# Autodesk Inventor assembly: アーム先端シールド1
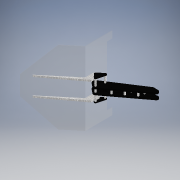
[picture p0: Inventor's stored thumbnail of the model, 180x180]
Saved by Autodesk Inventor 2020 (Build 240168000, 168)
## iProperties
Created: 2019-09-18
Part Number: アーム先端シールド1
Document SubType Name: Assembly
Designer: 雪村
Author: 雪村
## Documents named in this file (8)
- C:\Users\white\Documents\SRDC\SRDC\Inventor_2017\2018年機体\2020年4年機体\アーム先端シールド1.iam
- C:\Users\white\Documents\SRDC\SRDC\Inventor_2017\2018年機体\2020年4年機体\アーム先端第1関節2.1.ipt
- C:\Users\white\Documents\SRDC\SRDC\Inventor_2017\2018年機体\2020年4年機体\アーム先端第1関節2.1_MIR.ipt
- C:\Users\white\Documents\SRDC\SRDC\Inventor_2017\2018年機体\パーツ\スペーサーm3,16.ipt
- C:\Users\white\Documents\SRDC\SRDC\Inventor_2017\2018年機体\2020年4年機体\アームシールド根本1.ipt
- C:\Users\white\Documents\SRDC\SRDC\Inventor_2017\2018年機体\2020年4年機体\アームシールド2.ipt
- C:\Users\white\Documents\SRDC\SRDC\Inventor_2017\2018年機体\パーツ\スペーサーm3,25.ipt
- C:\Users\white\Documents\SRDC\SRDC\Inventor_2017\2018年機体\2020年4年機体\アーム抑えツイン1.ipt
## Components (22 placed, 7 different names)
1. アーム先端第1関節2.1:1 — 挿入:10, 挿入:11, 挿入:17, 挿入:18, 挿入:21
2. アーム先端第1関節2.1_MIR:1 — 挿入:1, 挿入:2, 挿入:3, 挿入:4, 挿入:5, 挿入:6, 挿入:7, 挿入:8, 挿入:9, 挿入:16, 挿入:19, 挿入:20, 挿入:22
3. スペーサーm3,16:1 — 挿入:2
4. スペーサーm3,16:2 — 挿入:1, 挿入:10
5. スペーサーm3,16:3 — 挿入:3
6. スペーサーm3,16:4 — 挿入:4
7. スペーサーm3,16:5 — 挿入:5
8. スペーサーm3,16:6 — 挿入:7
9. スペーサーm3,16:7 — 挿入:8
10. スペーサーm3,16:8 — 挿入:9
11. スペーサーm3,16:9 — 挿入:6, 挿入:11
12. アームシールド根本1:1 — 挿入:14, 挿入:15
13. アームシールド2:1 — 挿入:12, 挿入:13, 挿入:14, 挿入:15
14. アームシールド根本1:2 — 挿入:12, 挿入:13, 挿入:16
15. スペーサーm3,25:1 — 挿入:17, 挿入:25
16. スペーサーm3,25:2 — 挿入:18
17. スペーサーm3,25:3 — 挿入:19, 挿入:23
18. スペーサーm3,25:4 — 挿入:20
19. スペーサーm3,25:5 — 挿入:22, 挿入:24
20. スペーサーm3,25:6 — 挿入:21, 挿入:26
21. アーム抑えツイン1:1 — 挿入:25, 挿入:26
22. アーム抑えツイン1:2 — 挿入:23, 挿入:24
## Relationships (26: Insert 26)
- 挿入:1 [Insert]: アーム先端第1関節2.1_MIR:1 ↔ スペーサーm3,16:2
- 挿入:2 [Insert]: アーム先端第1関節2.1_MIR:1 ↔ スペーサーm3,16:1
- 挿入:3 [Insert]: アーム先端第1関節2.1_MIR:1 ↔ スペーサーm3,16:3
- 挿入:4 [Insert]: アーム先端第1関節2.1_MIR:1 ↔ スペーサーm3,16:4
- 挿入:5 [Insert]: アーム先端第1関節2.1_MIR:1 ↔ スペーサーm3,16:5
- 挿入:6 [Insert]: アーム先端第1関節2.1_MIR:1 ↔ スペーサーm3,16:9
- 挿入:7 [Insert]: アーム先端第1関節2.1_MIR:1 ↔ スペーサーm3,16:6
- 挿入:8 [Insert]: アーム先端第1関節2.1_MIR:1 ↔ スペーサーm3,16:7
- 挿入:9 [Insert]: アーム先端第1関節2.1_MIR:1 ↔ スペーサーm3,16:8
- 挿入:10 [Insert]: アーム先端第1関節2.1:1 ↔ スペーサーm3,16:2
- 挿入:11 [Insert]: アーム先端第1関節2.1:1 ↔ スペーサーm3,16:9
- 挿入:12 [Insert]: アームシールド2:1 ↔ アームシールド根本1:2
- 挿入:13 [Insert]: アームシールド2:1 ↔ アームシールド根本1:2
- 挿入:14 [Insert]: アームシールド根本1:1 ↔ アームシールド2:1
- 挿入:15 [Insert]: アームシールド根本1:1 ↔ アームシールド2:1
- 挿入:16 [Insert] (18 mm): アーム先端第1関節2.1_MIR:1 ↔ アームシールド根本1:2
- 挿入:17 [Insert]: アーム先端第1関節2.1:1 ↔ スペーサーm3,25:1
- 挿入:18 [Insert]: アーム先端第1関節2.1:1 ↔ スペーサーm3,25:2
- 挿入:19 [Insert]: アーム先端第1関節2.1_MIR:1 ↔ スペーサーm3,25:3
- 挿入:20 [Insert]: アーム先端第1関節2.1_MIR:1 ↔ スペーサーm3,25:4
- 挿入:21 [Insert]: アーム先端第1関節2.1:1 ↔ スペーサーm3,25:6
- 挿入:22 [Insert]: アーム先端第1関節2.1_MIR:1 ↔ スペーサーm3,25:5
- 挿入:23 [Insert]: スペーサーm3,25:3 ↔ アーム抑えツイン1:2
- 挿入:24 [Insert]: スペーサーm3,25:5 ↔ アーム抑えツイン1:2
- 挿入:25 [Insert]: スペーサーm3,25:1 ↔ アーム抑えツイン1:1
- 挿入:26 [Insert]: スペーサーm3,25:6 ↔ アーム抑えツイン1:1
